# Autodesk Inventor assembly: Gimbal_v2
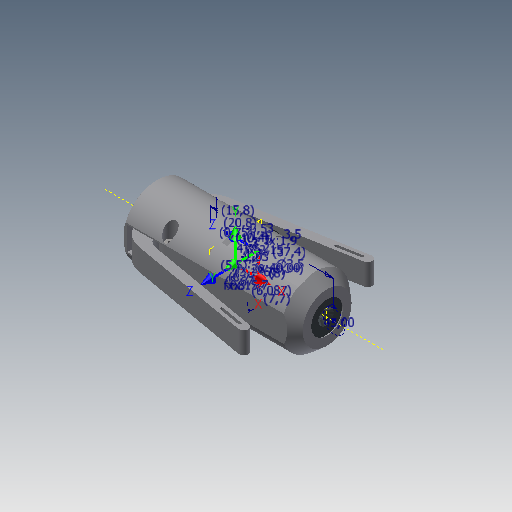
[picture p0: Inventor's stored thumbnail of the model, 512x512]
Saved by Autodesk Inventor 2021.4 (Build 254397000, 397)
## iProperties
Created: 2022-04-26
Part Number: Gimbal_v2
Material: Generisch
Document SubType Name: Assembly
Designer: alexw
Mass: 29.6625 g
Surface Area: 197.192 cm^2
Volume: 25.5218 cm^3
Density: 1.16224 g/cm^3
Author: alexw
## Documents named in this file (13)
- C:\Users\alexw\Documents\Inventor\Projects\03_CurrentProjects\MasterThesis\TrainingConsol_220422\Workgroups\Workgroup\Gimbal_v2.iam
- C:\Users\alexw\Documents\Inventor\Projects\03_CurrentProjects\MasterThesis\TrainingConsol_220422\Workgroups\Workgroup_new\GripperLever_v2.ipt
- C:\Users\alexw\Documents\Inventor\Projects\03_CurrentProjects\MasterThesis\TrainingConsol_220422\Workgroups\Workgroup_new\GripperLever_right_v2.ipt
- C:\Users\alexw\Documents\Inventor\Projects\03_CurrentProjects\MasterThesis\TrainingConsol_220422\Workgroups\Workgroup_new\Gimbal_Lower_Half.ipt
- C:\Users\alexw\Documents\Inventor\Projects\03_CurrentProjects\MasterThesis\TrainingConsol_220422\Workgroups\Workgroup_new\Gimbal_GripHalf_TopV2.ipt
- C:\Users\alexw\Documents\Inventor\Projects\03_CurrentProjects\MasterThesis\TrainingConsol_220422\Workgroups\Workgroup_new\Gimbal_GripHalf_BottomV2.ipt
- C:\Users\alexw\Documents\Inventor\Projects\03_CurrentProjects\MasterThesis\TrainingConsol_220422\Workgroups\Workgroup\ContentCenter\en-US\ISO 4762(2)\ISO 4762 - M2 x 10ISO.ipt
- C:\Users\alexw\Documents\Inventor\Projects\03_CurrentProjects\MasterThesis\TrainingConsol_220422\Workgroups\Workgroup_new\magnetic_annular_body_v2.ipt
- C:\Users\alexw\Documents\Inventor\Projects\03_CurrentProjects\MasterThesis\TrainingConsol_220422\Workgroups\Workgroup\Downloads\W 6173\SKF_W 617_3.iam
- C:\Users\alexw\Documents\Inventor\Projects\03_CurrentProjects\MasterThesis\TrainingConsol_220422\Workgroups\Workgroup_new\Gimbal_Lower_Half_Snapper.ipt
- C:\Users\alexw\Documents\Inventor\Projects\03_CurrentProjects\MasterThesis\TrainingConsol_220422\Workgroups\Workgroup\Gimbal_IMU_Sled_Assembly.iam
- C:\Users\alexw\Documents\Inventor\Projects\03_CurrentProjects\MasterThesis\TrainingConsol_220422\Workgroups\Workgroup\HallSensorMagnet.ipt
- C:\Users\alexw\Documents\Inventor\Projects\03_CurrentProjects\MasterThesis\TrainingConsol_220422\Workgroups\Workgroup\Shaft_3x17.ipt
## Components (18 placed, 12 different names)
1. Gimbal_GripHalf_BottomV2:1 — Flush:1, Flush:2, Flush:3, Mate:12, Mate:18, Mate:20, Mate:22, Mate:26, Mate:54, Mate:56, Mate:59, Mate:64
2. Gimbal_GripHalf_TopV2:1 — Flush:4, Flush:5, Flush:6, Mate:11, Flush:9, Mate:19, Mate:21, Mate:53, Mate:57, Mate:58, Mate:63, Mate:65
3. GripperLever_v2:1 — Mate:26, Flush:11, Rotation:1, Mate:61, Flush:12
4. GripperLever_right_v2:1 — Mate:22, Flush:11, Mate:53, Rotation:1, Mate:62, Angle:1
5. Gimbal_IMU_Sled_Assembly:1 [sub-assembly] — Mate:56, Mate:59, Mate:60
6. Gimbal_Lower_Half:1 — Mate:11, Flush:9, Mate:12, Mate:36, Mate:37, Mate:45, Mate:46, Mate:49, Mate:50, Mate:51, Mate:52, Angle:1
7. ISO 4762 M2 x 10:1 — Mate:18, Mate:19
8. ISO 4762 M2 x 10:2 — Mate:20, Mate:21
9. SKF_W 617_3:1 [sub-assembly]
10. SKF_W 617_3:2 [sub-assembly]
11. SKF_W 617_3:3 [sub-assembly] — Mate:58
12. SKF_W 617_3:4 [sub-assembly] — Mate:57
13. magnetic_annular_body_v2:1 — Mate:36, Mate:37
14. Gimbal_Lower_Half_Snapper:1 — Mate:45, Mate:46, Mate:51
15. Gimbal_Lower_Half_Snapper:2 — Mate:49, Mate:50, Mate:52
16. HallSensorMagnet:1 — Mate:61, Flush:12
17. Shaft_3x17:1 — Mate:62, Mate:63
18. Shaft_3x17:2 — Mate:64, Mate:65
## Relationships (44: Mate 33, Flush 9, RelateRotation 1, Angle 1)
- Flush:1: Gimbal_GripHalf_BottomV2:1
- Flush:2: Gimbal_GripHalf_BottomV2:1
- Flush:3: Gimbal_GripHalf_BottomV2:1
- Flush:4: Gimbal_GripHalf_TopV2:1
- Flush:5: Gimbal_GripHalf_TopV2:1
- Flush:6: Gimbal_GripHalf_TopV2:1
- Mate:11: Gimbal_GripHalf_TopV2:1 ↔ Gimbal_Lower_Half:1
- Flush:9: Gimbal_GripHalf_TopV2:1 ↔ Gimbal_Lower_Half:1
- Mate:12: Gimbal_GripHalf_BottomV2:1 ↔ Gimbal_Lower_Half:1
- Mate:18: Gimbal_GripHalf_BottomV2:1 ↔ ISO 4762 M2 x 10:1
- Mate:19: Gimbal_GripHalf_TopV2:1 ↔ ISO 4762 M2 x 10:1
- Mate:20: Gimbal_GripHalf_BottomV2:1 ↔ ISO 4762 M2 x 10:2
- Mate:21: Gimbal_GripHalf_TopV2:1 ↔ ISO 4762 M2 x 10:2
- Mate:22 (0.4 mm): Gimbal_GripHalf_BottomV2:1 ↔ GripperLever_right_v2:1
- Mate:26: Gimbal_GripHalf_BottomV2:1 ↔ GripperLever_v2:1
- [Mate]: Gimbal_GripHalf_BottomV2:1 ↔ SKF_W 617_3:2
- [Mate]: Gimbal_GripHalf_BottomV2:1 ↔ SKF_W 617_3:1
- [Mate]: Gimbal_GripHalf_TopV2:1 ↔ SKF_W 617_3:4
- [Mate]: Gimbal_GripHalf_TopV2:1 ↔ SKF_W 617_3:3
- Mate:36: Gimbal_Lower_Half:1 ↔ magnetic_annular_body_v2:1
- Mate:37: Gimbal_Lower_Half:1 ↔ magnetic_annular_body_v2:1
- [Mate]: Gimbal_GripHalf_BottomV2:1 ↔ SKF_W 617_3:2
- Mate:45: Gimbal_Lower_Half:1 ↔ Gimbal_Lower_Half_Snapper:1
- Mate:46: Gimbal_Lower_Half:1 ↔ Gimbal_Lower_Half_Snapper:1
- Mate:49: Gimbal_Lower_Half:1 ↔ Gimbal_Lower_Half_Snapper:2
- Mate:50: Gimbal_Lower_Half:1 ↔ Gimbal_Lower_Half_Snapper:2
- Mate:51: Gimbal_Lower_Half:1 ↔ Gimbal_Lower_Half_Snapper:1
- Mate:52: Gimbal_Lower_Half:1 ↔ Gimbal_Lower_Half_Snapper:2
- Flush:11: GripperLever_v2:1 ↔ GripperLever_right_v2:1
- Mate:53: Gimbal_GripHalf_TopV2:1 ↔ GripperLever_right_v2:1
- Rotation:1 [RelateRotation] (1 ul): GripperLever_v2:1 ↔ GripperLever_right_v2:1
- Mate:54: Gimbal_GripHalf_BottomV2:1
- Mate:56: Gimbal_GripHalf_BottomV2:1 ↔ Gimbal_IMU_Sled_Assembly:1
- Mate:57: Gimbal_GripHalf_TopV2:1 ↔ SKF_W 617_3:4
- Mate:58: Gimbal_GripHalf_TopV2:1 ↔ SKF_W 617_3:3
- Mate:59: Gimbal_GripHalf_BottomV2:1 ↔ Gimbal_IMU_Sled_Assembly:1
- Mate:60: Gimbal_IMU_Sled_Assembly:1
- Mate:61: GripperLever_v2:1 ↔ HallSensorMagnet:1
- Flush:12: GripperLever_v2:1 ↔ HallSensorMagnet:1
- Mate:62: GripperLever_right_v2:1 ↔ Shaft_3x17:1
- Mate:63: Gimbal_GripHalf_TopV2:1 ↔ Shaft_3x17:1
- Mate:64: Gimbal_GripHalf_BottomV2:1 ↔ Shaft_3x17:2
- Mate:65: Gimbal_GripHalf_TopV2:1 ↔ Shaft_3x17:2
- Angle:1 (190 deg): GripperLever_right_v2:1 ↔ Gimbal_Lower_Half:1
